# Autodesk Inventor assembly: Clutch Concept
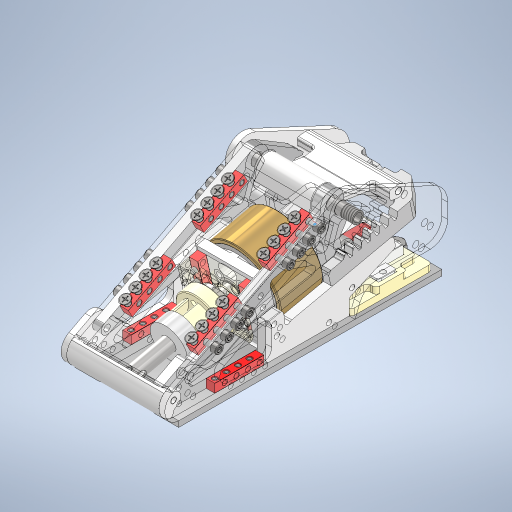
[picture p0: Inventor's stored thumbnail of the model, 512x512]
Saved by Autodesk Inventor 2023.4 (Build 274418000, 418)
## iProperties
Created: 2024-02-03
Part Number: Clutch Concept
Document SubType Name: Assembly
Designer: Nathan Cai
Mass: 541.92 g
Surface Area: 1727.46 cm^2
Volume: 204.134 cm^3
Density: 2.65472 g/cm^3
Author: Nathan Cai
## Documents named in this file (42)
- E:\Documents\Inventor\Bleep V1.2\Clutch Concept.iam
- E:\Documents\Inventor\Bleep V1.2\Flywheel.ipt
- E:\Documents\Inventor\Bleep V1.2\Thrust Bearing.ipt
- E:\Documents\Inventor\Bleep V1.2\BB 13x19x4.ipt
- E:\Documents\Inventor\Bleep V1.2\Cup.ipt
- E:\Documents\Inventor\Bleep V1.2\1561T741_Stacked Wave Disc Spring\1561T741_Stacked Wave Disc Spring.ipt
- E:\Documents\Inventor\Bleep V1.2\AKK RS2205 2300KV\AKK RS2205 2300KV.iam
- E:\Documents\Inventor\Bleep V1.2\Nut Strip 2x1 - 4-40.ipt
- E:\Documents\Inventor\Bleep V1.2\BB 37mm x 30mm x 4mm.ipt
- E:\Documents\Inventor\Bleep V1.2\Motor Plate.ipt
- E:\Documents\Inventor\Bleep V1.2\Uprights.ipt
- E:\Documents\Inventor\Bleep V1.2\Nut Strip 4x4 - 4-40.ipt
- E:\Documents\Inventor\Bleep V1.2\5172T23_Metal Gear - 20 Degree Pressure Angle\5172T23_Metal Gear - 20 Degree Pressure Angle.ipt
- E:\Documents\Inventor\Bleep V1.2\BB .25x.5x.1875 - Flangeless.ipt
- E:\Documents\Inventor\Content Center Files\R2023\en-US\ANSI B18.3(13)\ANSI B18.3 - 4-40 UNC - 0.375(22).ipt
- E:\Documents\Inventor\Bleep V1.2\Lever.ipt
- E:\Documents\Inventor\Bleep V1.2\Servo Support.ipt
- E:\Documents\Inventor\Bleep V1.2\Part1\Part1.ipt
- E:\Documents\Inventor\Bleep V1.2\Cam - Lever.ipt
- E:\Documents\Inventor\Bleep V1.2\Cam - Shell.ipt
- E:\Documents\Inventor\Bleep V1.2\BB 3x7x3.ipt
- E:\Documents\Inventor\Bleep V1.2\Ramp.ipt
- E:\Documents\Inventor\Bleep V1.2\Lever - Copy.ipt
- E:\Documents\Inventor\Bleep V1.2\Brace.ipt
- E:\Documents\Inventor\Bleep V1.2\BB 3x7x3 - Copy.ipt
- E:\Documents\Inventor\Bleep V1.2\Shaft - Arms.ipt
- E:\Documents\Inventor\Bleep V1.2\Shaft - Flywheel C.ipt
- E:\Documents\Inventor\Bleep V1.2\Clutch C.ipt
- E:\Documents\Inventor\Bleep V1.2\Spring Mount.ipt
- E:\Documents\Inventor\Bleep V1.2\Spring Spool.ipt
- E:\Documents\Inventor\Bleep V1.2\Collar.ipt
- E:\Documents\Inventor\Bleep V1.2\Bottom Plate.ipt
- E:\Documents\Inventor\Content Center Files\R2023\en-US\ANSI B18.6.3(12)\ANSI B18.6.3 - 4-40 UNC - 0.375(15_).ipt
- E:\Documents\Inventor\Bleep V1.2\Crown.ipt
- E:\Documents\Inventor\Bleep V1.2\Front Bumper.ipt
- E:\Documents\Inventor\Content Center Files\R2023\en-US\ANSI B18.6.3(12)\ANSI B18.6.3 - 4-40 UNC - 0.3125(15_).ipt
- E:\Documents\Inventor\Content Center Files\R2023\en-US\ANSI B18.6.3(12)\ANSI B18.6.3 - 6-32 UNC - 0.375(15_).ipt
- E:\Documents\Inventor\Content Center Files\R2023\en-US\ANSI B18.2.2(06)\ANSI B18.2.2 - 6 - 32(06).ipt
- E:\Documents\Inventor\Content Center Files\R2023\en-US\ANSI B18.6.3(14)\ANSI B18.6.3 - 6-32 UNC - 0.625(6).ipt
- E:\Documents\Inventor\Bleep V1.2\Rack - Slot.ipt
- E:\Documents\Inventor\Bleep V1.2\Export\STL\Lever Spacer.ipt
- E:\Documents\Inventor\Bleep V1.2\Uprights- Exterior.ipt
## Components (110 placed, 41 different names)
1. Front Bumper:1 — Angle:5
2. Bottom Plate:1 — Mate:347, Flush:153, Mate:402, Mate:403, Mate:404, Mate:405, Mate:406, Mate:407, Mate:408, Mate:409, Mate:410, Mate:411, Mate:412, Mate:413, Mate:414, Mate:415, Mate:416, Mate:417, Mate:418, Mate:420, Mate:422, Mate:424
3. Crown:1 — Mate:386, Mate:387
4. Lever Spacer:1 — Mate:462, Mate:463
5. Uprights- Exterior:1 — Mate:470, Mate:471, Mate:472
6. Uprights- Exterior:2 — Mate:473, Mate:474, Mate:475
7. Flywheel:1 — Mate:37, Flush:102, Mate:104, Mate:105, Mate:275, Mate:309
8. Shaft - Flywheel C:1 — Mate:306, Mate:307, Mate:308, Mate:310, Mate:311, Mate:312, Mate:313, Mate:314, Mate:315, Angle:4, Mate:319, Mate:321, Mate:324
9. Shaft - Arms:1 — Mate:257, Flush:118, Mate:386, Mate:471, Mate:474
10. Clutch C:1 — Mate:308, Angle:4
11. Rack - Slot:1 — Angle:1, Angle:3, Rotation/Translation:1, Mate:315, Mate:313, Mate:314
12. Cup:1 — Mate:26, Mate:27, Angle:1, Tangent:1
13. AKK RS2205 2300KV:1 [sub-assembly] — Mate:37, Flush:102, Mate:426
14. Motor Plate:1 — Mate:106, Mate:107, Mate:128, Mate:129, Mate:131, Mate:132, Mate:134, Mate:136, Flush:106, Mate:144, Mate:145, Mate:146, Mate:147, Mate:148, Mate:149, Mate:150, Mate:151, Mate:152, Mate:153, Mate:154, Mate:155, Mate:156, Mate:157, Mate:158, Mate:159, Flush:149, Mate:426
15. 1561T741_Stacked Wave Disc Spring:1 — Mate:311, Mate:312
16. Spring Mount:1 — Mate:316, Flush:149, Mate:317, Mate:320
17. Thrust Bearing:1 — Mate:319, Mate:320, Mate:322
18. Spring Spool:1 — Mate:321, Mate:322, Mate:325
19. Collar:1 — Mate:324, Mate:325
20. Uprights:1 — Mate:128, Mate:130, Flush:103, Flush:104, Mate:133, Mate:138, Mate:141, Flush:107, Mate:168, Mate:169, Flush:108, Mate:229, Mate:230, Flush:110, Mate:257, Mate:266, Mate:267, Mate:268, Mate:269, Flush:125, Mate:317, Mate:289, Mate:347, Mate:363
21. Uprights:2 — Flush:103, Mate:132, Flush:104, Mate:135, Mate:137, Mate:139, Mate:140, Mate:191, Mate:226, Mate:228, Flush:111, Mate:263, Mate:264, Mate:270, Mate:271, Flush:124, Mate:292, Mate:362, Mate:387, Angle:5
22. Brace:1 — Mate:226, Mate:228, Flush:111, Mate:292, Mate:470
23. Brace:2 — Mate:229, Mate:230, Flush:110, Mate:289, Mate:473
24. Nut Strip 4x4 - 4-40:1 — Mate:129, Mate:130, Mate:131, Mate:133, Mate:316
25. Nut Strip 4x4 - 4-40:2 — Mate:134, Mate:135, Mate:136, Mate:137
26. 5172T23_Metal Gear - 20 Degree Pressure Angle:1 — Mate:138, Mate:141, Flush:105, Angle:3, Mate:198, Mate:199, Mate:200, Mate:201, Mate:202, Mate:203, Mate:204, Rotation/Translation:1, Flush:118, Mate:369, Mate:427, Mate:428, Mate:429, Mate:430, Mate:431, Mate:432, Mate:433, Mate:434, Mate:435, Mate:436, Mate:437, Mate:438, Mate:439, Mate:440, Mate:441, Mate:442
27. 5172T23_Metal Gear - 20 Degree Pressure Angle:2 — Mate:139, Mate:140, Flush:105, Mate:192, Mate:193, Mate:194, Mate:195, Mate:196, Mate:197, Flush:150, Mate:443, Mate:444, Mate:445, Mate:446, Mate:447, Mate:448, Mate:449, Mate:450, Mate:451, Mate:452, Mate:453, Mate:454, Mate:455, Mate:456, Mate:457, Mate:458
28. BB .25x.5x.1875 - Flangeless:1 — Flush:106, Mate:310
29. Lever:1 — Mate:168, Mate:169, Tangent:1, Mate:181, Mate:182, Mate:190, Mate:326, Mate:327
30. Lever - Copy:1
31. Part1:1 — Mate:179, Mate:180, Mate:186, Mate:187, Mate:188
32. Cam - Lever:1 — Mate:177, Mate:178, Mate:327
33. Cam - Shell:1 — Mate:177, Mate:178, Mate:179, Mate:180
34. BB 3x7x3:1 — Mate:181, Mate:182
35. BB 3x7x3:2 — Mate:462, Mate:463
36. BB 3x7x3 - Copy:1 — Mate:190, Mate:326
37. BB 13x19x4:1 — Mate:26, Mate:27
38. BB 37mm x 30mm x 4mm:1 — Mate:104, Mate:105, Mate:106, Mate:107
39. BB .25x.5x.1875 - Flangeless:2 — Mate:275, Mate:306, Mate:307, Mate:309
40. Servo Support:1 — Mate:186, Mate:187, Mate:188, Flush:108, Mate:191, Flush:153, Mate:419, Mate:421, Mate:423, Mate:425
41. Ramp:1 — Mate:204, Flush:150, Mate:369, Mate:370, Mate:371, Mate:372, Mate:373, Mate:374, Mate:375, Mate:376, Mate:377, Mate:378, Mate:379, Mate:380, Mate:381, Mate:382, Mate:383, Mate:384, Mate:385
42. Nut Strip 4x4 - 4-40:3 — Mate:192, Mate:193, Mate:194
43. Nut Strip 4x4 - 4-40:5 — Mate:199, Mate:200, Mate:201
44. Nut Strip 4x4 - 4-40:6 — Mate:198, Mate:202, Mate:203
45. Nut Strip 4x4 - 4-40:7 — Mate:195, Mate:196, Mate:197
46. Nut Strip 4x4 - 4-40:8 — Mate:266, Mate:267, Mate:363, Mate:475
47. Nut Strip 4x4 - 4-40:9 — Mate:263, Mate:264, Mate:362, Mate:472
48. Nut Strip 2x1 - 4-40:3 — Mate:270, Mate:271, Flush:124
49. Nut Strip 2x1 - 4-40:4 — Mate:268, Mate:269, Flush:125
50. Cross Recessed Flat Countersunk Head Machine Screw - Type II - Inch 6-32 x 5/8:1
51. Spline Socket Head Cap Screw - Inch 4-40 UNC - 0.375:9 — Mate:427, Mate:428
52. Spline Socket Head Cap Screw - Inch 4-40 UNC - 0.375:10 — Mate:429, Mate:430
53. Spline Socket Head Cap Screw - Inch 4-40 UNC - 0.375:11 — Mate:431, Mate:432
54. Spline Socket Head Cap Screw - Inch 4-40 UNC - 0.375:12 — Mate:433, Mate:434
55. Spline Socket Head Cap Screw - Inch 4-40 UNC - 0.375:13 — Mate:435, Mate:436
56. Spline Socket Head Cap Screw - Inch 4-40 UNC - 0.375:14 — Mate:437, Mate:438
57. Spline Socket Head Cap Screw - Inch 4-40 UNC - 0.375:15 — Mate:439, Mate:440
58. Spline Socket Head Cap Screw - Inch 4-40 UNC - 0.375:16 — Mate:441, Mate:442
59. Spline Socket Head Cap Screw - Inch 4-40 UNC - 0.375:17 — Mate:443, Mate:444
60. Spline Socket Head Cap Screw - Inch 4-40 UNC - 0.375:18 — Mate:445, Mate:446
61. Spline Socket Head Cap Screw - Inch 4-40 UNC - 0.375:19 — Mate:447, Mate:448
62. Spline Socket Head Cap Screw - Inch 4-40 UNC - 0.375:20 — Mate:449, Mate:450
63. Spline Socket Head Cap Screw - Inch 4-40 UNC - 0.375:21 — Mate:451, Mate:452
64. Spline Socket Head Cap Screw - Inch 4-40 UNC - 0.375:22 — Mate:453, Mate:454
65. Spline Socket Head Cap Screw - Inch 4-40 UNC - 0.375:23 — Mate:455, Mate:456
66. Spline Socket Head Cap Screw - Inch 4-40 UNC - 0.375:24 — Mate:457, Mate:458
67. Cross Recessed Flat Countersunk Head Machine Screw - Type I - Inch 4-40 x 5/16:1 — Mate:402
68. Cross Recessed Flat Countersunk Head Machine Screw - Type I - Inch 4-40 x 5/16:2 — Mate:403
69. Cross Recessed Flat Countersunk Head Machine Screw - Type I - Inch 4-40 x 5/16:3 — Mate:404
70. Cross Recessed Flat Countersunk Head Machine Screw - Type I - Inch 4-40 x 5/16:4 — Mate:405
71. Cross Recessed Flat Countersunk Head Machine Screw - Type I - Inch 4-40 x 5/16:5 — Mate:406
72. Cross Recessed Flat Countersunk Head Machine Screw - Type I - Inch 4-40 x 5/16:6 — Mate:407
73. Cross Recessed Flat Countersunk Head Machine Screw - Type I - Inch 4-40 x 5/16:7 — Mate:408
74. Cross Recessed Flat Countersunk Head Machine Screw - Type I - Inch 4-40 x 5/16:8 — Mate:409
75. Cross Recessed Flat Countersunk Head Machine Screw - Type I - Inch 4-40 x 5/16:9 — Mate:410
76. Cross Recessed Flat Countersunk Head Machine Screw - Type I - Inch 4-40 x 5/16:10 — Mate:411
77. Cross Recessed Flat Countersunk Head Machine Screw - Type I - Inch 4-40 x 5/16:11 — Mate:412
78. Cross Recessed Flat Countersunk Head Machine Screw - Type I - Inch 4-40 x 5/16:12 — Mate:413
79. Cross Recessed Flat Countersunk Head Machine Screw - Type I - Inch 6-32 x 3/8:1 — Mate:414
80. Hex Machine Screw Nut - Inch 6 - 32:1 — Mate:418, Mate:419
81. Cross Recessed Flat Countersunk Head Machine Screw - Type I - Inch 6-32 x 3/8:2 — Mate:415
82. Cross Recessed Flat Countersunk Head Machine Screw - Type I - Inch 6-32 x 3/8:3 — Mate:416
83. Cross Recessed Flat Countersunk Head Machine Screw - Type I - Inch 6-32 x 3/8:4 — Mate:417
84. Hex Machine Screw Nut - Inch 6 - 32:2 — Mate:420, Mate:421
85. Hex Machine Screw Nut - Inch 6 - 32:3 — Mate:422, Mate:423
86. Hex Machine Screw Nut - Inch 6 - 32:4 — Mate:424, Mate:425
87. Cross Recessed Flat Countersunk Head Machine Screw - Type I - Inch 4-40 x 3/8:1 — Mate:370
88. Cross Recessed Flat Countersunk Head Machine Screw - Type I - Inch 4-40 x 3/8:2 — Mate:371
89. Cross Recessed Flat Countersunk Head Machine Screw - Type I - Inch 4-40 x 3/8:3 — Mate:372
90. Cross Recessed Flat Countersunk Head Machine Screw - Type I - Inch 4-40 x 3/8:4 — Mate:373
91. Cross Recessed Flat Countersunk Head Machine Screw - Type I - Inch 4-40 x 3/8:5 — Mate:374
92. Cross Recessed Flat Countersunk Head Machine Screw - Type I - Inch 4-40 x 3/8:6 — Mate:375
93. Cross Recessed Flat Countersunk Head Machine Screw - Type I - Inch 4-40 x 3/8:7 — Mate:376
94. Cross Recessed Flat Countersunk Head Machine Screw - Type I - Inch 4-40 x 3/8:8 — Mate:377
95. Cross Recessed Flat Countersunk Head Machine Screw - Type I - Inch 4-40 x 3/8:9 — Mate:378
96. Cross Recessed Flat Countersunk Head Machine Screw - Type I - Inch 4-40 x 3/8:10 — Mate:379
97. Cross Recessed Flat Countersunk Head Machine Screw - Type I - Inch 4-40 x 3/8:11 — Mate:380
98. Cross Recessed Flat Countersunk Head Machine Screw - Type I - Inch 4-40 x 3/8:12 — Mate:381
99. Cross Recessed Flat Countersunk Head Machine Screw - Type I - Inch 4-40 x 3/8:13 — Mate:382
100. Cross Recessed Flat Countersunk Head Machine Screw - Type I - Inch 4-40 x 3/8:14 — Mate:383
101. Cross Recessed Flat Countersunk Head Machine Screw - Type I - Inch 4-40 x 3/8:15 — Mate:384
102. Cross Recessed Flat Countersunk Head Machine Screw - Type I - Inch 4-40 x 3/8:16 — Mate:385
103. Spline Socket Head Cap Screw - Inch 4-40 UNC - 0.375:1 — Mate:144, Mate:145
104. Spline Socket Head Cap Screw - Inch 4-40 UNC - 0.375:2 — Mate:146, Mate:147
105. Spline Socket Head Cap Screw - Inch 4-40 UNC - 0.375:3 — Mate:148, Mate:149
106. Spline Socket Head Cap Screw - Inch 4-40 UNC - 0.375:4 — Mate:150, Mate:151
107. Spline Socket Head Cap Screw - Inch 4-40 UNC - 0.375:5 — Mate:152, Mate:153
108. Spline Socket Head Cap Screw - Inch 4-40 UNC - 0.375:6 — Mate:154, Mate:155
109. Spline Socket Head Cap Screw - Inch 4-40 UNC - 0.375:7 — Mate:156, Mate:157
110. Spline Socket Head Cap Screw - Inch 4-40 UNC - 0.375:8 — Mate:158, Mate:159
## Relationships (214: Mate 193, Flush 15, Angle 4, Tangent 1, RelateRotateTranslate 1)
- [Mate]: Clutch C:1 ↔ BB 13x19x4:1
- [Mate]: Clutch C:1 ↔ BB 13x19x4:1
- Mate:26: Cup:1 ↔ BB 13x19x4:1
- Mate:27: Cup:1 ↔ BB 13x19x4:1
- Mate:37: Flywheel:1 ↔ AKK RS2205 2300KV:1
- Angle:1 (0 deg): Rack - Slot:1 ↔ Cup:1
- Flush:102: Flywheel:1 ↔ AKK RS2205 2300KV:1
- Mate:104: Flywheel:1 ↔ BB 37mm x 30mm x 4mm:1
- Mate:105: Flywheel:1 ↔ BB 37mm x 30mm x 4mm:1
- Mate:106: Motor Plate:1 ↔ BB 37mm x 30mm x 4mm:1
- Mate:107: Motor Plate:1 ↔ BB 37mm x 30mm x 4mm:1
- Mate:128: Motor Plate:1 ↔ Uprights:1
- Mate:129: Motor Plate:1 ↔ Nut Strip 4x4 - 4-40:1
- Mate:130: Uprights:1 ↔ Nut Strip 4x4 - 4-40:1
- Mate:131: Motor Plate:1 ↔ Nut Strip 4x4 - 4-40:1
- Flush:103: Uprights:1 ↔ Uprights:2
- Mate:132: Motor Plate:1 ↔ Uprights:2
- Flush:104: Uprights:1 ↔ Uprights:2
- Mate:133: Uprights:1 ↔ Nut Strip 4x4 - 4-40:1
- Mate:134: Motor Plate:1 ↔ Nut Strip 4x4 - 4-40:2
- Mate:135: Uprights:2 ↔ Nut Strip 4x4 - 4-40:2
- Mate:136: Motor Plate:1 ↔ Nut Strip 4x4 - 4-40:2
- Mate:137: Uprights:2 ↔ Nut Strip 4x4 - 4-40:2
- Mate:138: Uprights:1 ↔ 5172T23_Metal Gear - 20 Degree Pressure Angle:1
- Mate:139: Uprights:2 ↔ 5172T23_Metal Gear - 20 Degree Pressure Angle:2
- Mate:140: Uprights:2 ↔ 5172T23_Metal Gear - 20 Degree Pressure Angle:2
- Mate:141: Uprights:1 ↔ 5172T23_Metal Gear - 20 Degree Pressure Angle:1
- Flush:105: 5172T23_Metal Gear - 20 Degree Pressure Angle:1 ↔ 5172T23_Metal Gear - 20 Degree Pressure Angle:2
- Flush:106: Motor Plate:1 ↔ BB .25x.5x.1875 - Flangeless:1
- Mate:144: Motor Plate:1 ↔ Spline Socket Head Cap Screw - Inch 4-40 UNC - 0.375:1
- Mate:145: Motor Plate:1 ↔ Spline Socket Head Cap Screw - Inch 4-40 UNC - 0.375:1
- Mate:146: Motor Plate:1 ↔ Spline Socket Head Cap Screw - Inch 4-40 UNC - 0.375:2
- Mate:147: Motor Plate:1 ↔ Spline Socket Head Cap Screw - Inch 4-40 UNC - 0.375:2
- Mate:148: Motor Plate:1 ↔ Spline Socket Head Cap Screw - Inch 4-40 UNC - 0.375:3
- Mate:149: Motor Plate:1 ↔ Spline Socket Head Cap Screw - Inch 4-40 UNC - 0.375:3
- Mate:150: Motor Plate:1 ↔ Spline Socket Head Cap Screw - Inch 4-40 UNC - 0.375:4
- Mate:151: Motor Plate:1 ↔ Spline Socket Head Cap Screw - Inch 4-40 UNC - 0.375:4
- Mate:152: Motor Plate:1 ↔ Spline Socket Head Cap Screw - Inch 4-40 UNC - 0.375:5
- Mate:153: Motor Plate:1 ↔ Spline Socket Head Cap Screw - Inch 4-40 UNC - 0.375:5
- Mate:154: Motor Plate:1 ↔ Spline Socket Head Cap Screw - Inch 4-40 UNC - 0.375:6
- Mate:155: Motor Plate:1 ↔ Spline Socket Head Cap Screw - Inch 4-40 UNC - 0.375:6
- Mate:156: Motor Plate:1 ↔ Spline Socket Head Cap Screw - Inch 4-40 UNC - 0.375:7
- Mate:157: Motor Plate:1 ↔ Spline Socket Head Cap Screw - Inch 4-40 UNC - 0.375:7
- Mate:158: Motor Plate:1 ↔ Spline Socket Head Cap Screw - Inch 4-40 UNC - 0.375:8
- Mate:159: Motor Plate:1 ↔ Spline Socket Head Cap Screw - Inch 4-40 UNC - 0.375:8
- Flush:107: Uprights:1
- Mate:168: Uprights:1 ↔ Lever:1
- Mate:169: Uprights:1 ↔ Lever:1
- Tangent:1: Cup:1 ↔ Lever:1
- Angle:3 (0 deg): Rack - Slot:1 ↔ 5172T23_Metal Gear - 20 Degree Pressure Angle:1
- [Mate]: Uprights:2 ↔ Lever - Copy:1
- [Mate]: Uprights:2 ↔ Lever - Copy:1
- [Mate]: Lever:1 ↔ Lever - Copy:1
- Mate:177: Cam - Lever:1 ↔ Cam - Shell:1
- Mate:178: Cam - Lever:1 ↔ Cam - Shell:1
- Mate:179: Part1:1 ↔ Cam - Shell:1
- Mate:180: Part1:1 ↔ Cam - Shell:1
- Mate:181: Lever:1 ↔ BB 3x7x3:1
- Mate:182: Lever:1 ↔ BB 3x7x3:1
- [Mate]: Lever - Copy:1 ↔ BB 3x7x3:2
- [Mate]: Lever - Copy:1 ↔ BB 3x7x3:2
- Mate:186: Part1:1 ↔ Servo Support:1
- Mate:187: Part1:1 ↔ Servo Support:1
- Mate:188: Part1:1 ↔ Servo Support:1
- Flush:108: Uprights:1 ↔ Servo Support:1
- Mate:190: Lever:1 ↔ BB 3x7x3 - Copy:1
- Mate:191: Uprights:2 ↔ Servo Support:1
- Mate:192: 5172T23_Metal Gear - 20 Degree Pressure Angle:2 ↔ Nut Strip 4x4 - 4-40:3
- Mate:193: 5172T23_Metal Gear - 20 Degree Pressure Angle:2 ↔ Nut Strip 4x4 - 4-40:3
- Mate:194: 5172T23_Metal Gear - 20 Degree Pressure Angle:2 ↔ Nut Strip 4x4 - 4-40:3
- Mate:195: 5172T23_Metal Gear - 20 Degree Pressure Angle:2 ↔ Nut Strip 4x4 - 4-40:7
- Mate:196: 5172T23_Metal Gear - 20 Degree Pressure Angle:2 ↔ Nut Strip 4x4 - 4-40:7
- Mate:197: 5172T23_Metal Gear - 20 Degree Pressure Angle:2 ↔ Nut Strip 4x4 - 4-40:7
- Mate:198: 5172T23_Metal Gear - 20 Degree Pressure Angle:1 ↔ Nut Strip 4x4 - 4-40:6
- Mate:199: 5172T23_Metal Gear - 20 Degree Pressure Angle:1 ↔ Nut Strip 4x4 - 4-40:5
- Mate:200: 5172T23_Metal Gear - 20 Degree Pressure Angle:1 ↔ Nut Strip 4x4 - 4-40:5
- Mate:201: 5172T23_Metal Gear - 20 Degree Pressure Angle:1 ↔ Nut Strip 4x4 - 4-40:5
- Mate:202: 5172T23_Metal Gear - 20 Degree Pressure Angle:1 ↔ Nut Strip 4x4 - 4-40:6
- Mate:203: 5172T23_Metal Gear - 20 Degree Pressure Angle:1 ↔ Nut Strip 4x4 - 4-40:6
- Mate:204: 5172T23_Metal Gear - 20 Degree Pressure Angle:1 ↔ Ramp:1
- Flush:150: 5172T23_Metal Gear - 20 Degree Pressure Angle:2 ↔ Ramp:1
- Mate:226: Uprights:2 ↔ Brace:1
- Mate:228: Uprights:2 ↔ Brace:1
- Mate:229: Uprights:1 ↔ Brace:2
- Mate:230: Uprights:1 ↔ Brace:2
- Rotation/Translation:1 [RelateRotateTranslate] (159.5929 mm): Rack - Slot:1 ↔ 5172T23_Metal Gear - 20 Degree Pressure Angle:1
- Flush:110: Uprights:1 ↔ Brace:2
- Flush:111: Uprights:2 ↔ Brace:1
- Mate:257: Shaft - Arms:1 ↔ Uprights:1
- Flush:118 (-6.35 mm): Shaft - Arms:1 ↔ 5172T23_Metal Gear - 20 Degree Pressure Angle:1
- Mate:315 (31.75 mm): Shaft - Flywheel C:1 ↔ Rack - Slot:1
- Mate:263: Uprights:2 ↔ Nut Strip 4x4 - 4-40:9
- Mate:264: Uprights:2 ↔ Nut Strip 4x4 - 4-40:9
- Mate:266: Uprights:1 ↔ Nut Strip 4x4 - 4-40:8
- Mate:267: Uprights:1 ↔ Nut Strip 4x4 - 4-40:8
- Mate:268: Uprights:1 ↔ Nut Strip 2x1 - 4-40:4
- Mate:269: Uprights:1 ↔ Nut Strip 2x1 - 4-40:4
- Mate:270: Uprights:2 ↔ Nut Strip 2x1 - 4-40:3
- Mate:271: Uprights:2 ↔ Nut Strip 2x1 - 4-40:3
- Flush:124: Uprights:2 ↔ Nut Strip 2x1 - 4-40:3
- Flush:125: Uprights:1 ↔ Nut Strip 2x1 - 4-40:4
- Mate:275: Flywheel:1 ↔ BB .25x.5x.1875 - Flangeless:2
- Mate:289: Uprights:1 ↔ Brace:2
- Mate:292: Uprights:2 ↔ Brace:1
- Mate:306: Shaft - Flywheel C:1 ↔ BB .25x.5x.1875 - Flangeless:2
- Mate:307: Shaft - Flywheel C:1 ↔ BB .25x.5x.1875 - Flangeless:2
- Mate:308: Shaft - Flywheel C:1 ↔ Clutch C:1
- Mate:309: Flywheel:1 ↔ BB .25x.5x.1875 - Flangeless:2
- Mate:310: Shaft - Flywheel C:1 ↔ BB .25x.5x.1875 - Flangeless:1
- Mate:311: Shaft - Flywheel C:1 ↔ 1561T741_Stacked Wave Disc Spring:1
- Mate:312: Shaft - Flywheel C:1 ↔ 1561T741_Stacked Wave Disc Spring:1
- Mate:313: Shaft - Flywheel C:1 ↔ Rack - Slot:1
- Mate:314: Shaft - Flywheel C:1 ↔ Rack - Slot:1
- Angle:4 (0 deg): Shaft - Flywheel C:1 ↔ Clutch C:1
- Mate:316: Spring Mount:1 ↔ Nut Strip 4x4 - 4-40:1
- Flush:149 (2.3813 mm): Motor Plate:1 ↔ Spring Mount:1
- Mate:317: Spring Mount:1 ↔ Uprights:1
- Mate:319: Shaft - Flywheel C:1 ↔ Thrust Bearing:1
- Mate:320: Spring Mount:1 ↔ Thrust Bearing:1
- Mate:321: Shaft - Flywheel C:1 ↔ Spring Spool:1
- Mate:322: Thrust Bearing:1 ↔ Spring Spool:1
- Mate:324: Shaft - Flywheel C:1 ↔ Collar:1
- Mate:325: Spring Spool:1 ↔ Collar:1
- Mate:326: Lever:1 ↔ BB 3x7x3 - Copy:1
- Mate:327: Lever:1 ↔ Cam - Lever:1
- Mate:347: Bottom Plate:1 ↔ Uprights:1
- Flush:153 (-3.175 mm): Bottom Plate:1 ↔ Servo Support:1
- Mate:362: Uprights:2 ↔ Nut Strip 4x4 - 4-40:9
- Mate:363: Uprights:1 ↔ Nut Strip 4x4 - 4-40:8
- Mate:369: 5172T23_Metal Gear - 20 Degree Pressure Angle:1 ↔ Ramp:1
- Mate:370: Ramp:1 ↔ Cross Recessed Flat Countersunk Head Machine Screw - Type I - Inch 4-40 x 3/8:1
- Mate:371: Ramp:1 ↔ Cross Recessed Flat Countersunk Head Machine Screw - Type I - Inch 4-40 x 3/8:2
- Mate:372: Ramp:1 ↔ Cross Recessed Flat Countersunk Head Machine Screw - Type I - Inch 4-40 x 3/8:3
- Mate:373: Ramp:1 ↔ Cross Recessed Flat Countersunk Head Machine Screw - Type I - Inch 4-40 x 3/8:4
- Mate:374: Ramp:1 ↔ Cross Recessed Flat Countersunk Head Machine Screw - Type I - Inch 4-40 x 3/8:5
- Mate:375: Ramp:1 ↔ Cross Recessed Flat Countersunk Head Machine Screw - Type I - Inch 4-40 x 3/8:6
- Mate:376: Ramp:1 ↔ Cross Recessed Flat Countersunk Head Machine Screw - Type I - Inch 4-40 x 3/8:7
- Mate:377: Ramp:1 ↔ Cross Recessed Flat Countersunk Head Machine Screw - Type I - Inch 4-40 x 3/8:8
- Mate:378: Ramp:1 ↔ Cross Recessed Flat Countersunk Head Machine Screw - Type I - Inch 4-40 x 3/8:9
- Mate:379: Ramp:1 ↔ Cross Recessed Flat Countersunk Head Machine Screw - Type I - Inch 4-40 x 3/8:10
- Mate:380: Ramp:1 ↔ Cross Recessed Flat Countersunk Head Machine Screw - Type I - Inch 4-40 x 3/8:11
- Mate:381: Ramp:1 ↔ Cross Recessed Flat Countersunk Head Machine Screw - Type I - Inch 4-40 x 3/8:12
- Mate:382: Ramp:1 ↔ Cross Recessed Flat Countersunk Head Machine Screw - Type I - Inch 4-40 x 3/8:13
- Mate:383: Ramp:1 ↔ Cross Recessed Flat Countersunk Head Machine Screw - Type I - Inch 4-40 x 3/8:14
- Mate:384: Ramp:1 ↔ Cross Recessed Flat Countersunk Head Machine Screw - Type I - Inch 4-40 x 3/8:15
- Mate:385: Ramp:1 ↔ Cross Recessed Flat Countersunk Head Machine Screw - Type I - Inch 4-40 x 3/8:16
- Mate:386: Crown:1 ↔ Shaft - Arms:1
- Mate:387: Crown:1 ↔ Uprights:2
- Angle:5 (180 deg): Front Bumper:1 ↔ Uprights:2
- Mate:402: Bottom Plate:1 ↔ Cross Recessed Flat Countersunk Head Machine Screw - Type I - Inch 4-40 x 5/16:1
- Mate:403: Bottom Plate:1 ↔ Cross Recessed Flat Countersunk Head Machine Screw - Type I - Inch 4-40 x 5/16:2
- Mate:404: Bottom Plate:1 ↔ Cross Recessed Flat Countersunk Head Machine Screw - Type I - Inch 4-40 x 5/16:3
- Mate:405: Bottom Plate:1 ↔ Cross Recessed Flat Countersunk Head Machine Screw - Type I - Inch 4-40 x 5/16:4
- Mate:406: Bottom Plate:1 ↔ Cross Recessed Flat Countersunk Head Machine Screw - Type I - Inch 4-40 x 5/16:5
- Mate:407: Bottom Plate:1 ↔ Cross Recessed Flat Countersunk Head Machine Screw - Type I - Inch 4-40 x 5/16:6
- Mate:408: Bottom Plate:1 ↔ Cross Recessed Flat Countersunk Head Machine Screw - Type I - Inch 4-40 x 5/16:7
- Mate:409: Bottom Plate:1 ↔ Cross Recessed Flat Countersunk Head Machine Screw - Type I - Inch 4-40 x 5/16:8
- Mate:410: Bottom Plate:1 ↔ Cross Recessed Flat Countersunk Head Machine Screw - Type I - Inch 4-40 x 5/16:9
- Mate:411: Bottom Plate:1 ↔ Cross Recessed Flat Countersunk Head Machine Screw - Type I - Inch 4-40 x 5/16:10
- Mate:412: Bottom Plate:1 ↔ Cross Recessed Flat Countersunk Head Machine Screw - Type I - Inch 4-40 x 5/16:11
- Mate:413: Bottom Plate:1 ↔ Cross Recessed Flat Countersunk Head Machine Screw - Type I - Inch 4-40 x 5/16:12
- Mate:414: Bottom Plate:1 ↔ Cross Recessed Flat Countersunk Head Machine Screw - Type I - Inch 6-32 x 3/8:1
- Mate:415: Bottom Plate:1 ↔ Cross Recessed Flat Countersunk Head Machine Screw - Type I - Inch 6-32 x 3/8:2
- Mate:416: Bottom Plate:1 ↔ Cross Recessed Flat Countersunk Head Machine Screw - Type I - Inch 6-32 x 3/8:3
- Mate:417: Bottom Plate:1 ↔ Cross Recessed Flat Countersunk Head Machine Screw - Type I - Inch 6-32 x 3/8:4
- Mate:418: Bottom Plate:1 ↔ Hex Machine Screw Nut - Inch 6 - 32:1
- Mate:419: Servo Support:1 ↔ Hex Machine Screw Nut - Inch 6 - 32:1
- Mate:420: Bottom Plate:1 ↔ Hex Machine Screw Nut - Inch 6 - 32:2
- Mate:421: Servo Support:1 ↔ Hex Machine Screw Nut - Inch 6 - 32:2
- Mate:422: Bottom Plate:1 ↔ Hex Machine Screw Nut - Inch 6 - 32:3
- Mate:423: Servo Support:1 ↔ Hex Machine Screw Nut - Inch 6 - 32:3
- Mate:424: Bottom Plate:1 ↔ Hex Machine Screw Nut - Inch 6 - 32:4
- Mate:425: Servo Support:1 ↔ Hex Machine Screw Nut - Inch 6 - 32:4
- Mate:426: AKK RS2205 2300KV:1 ↔ Motor Plate:1
- Mate:427: 5172T23_Metal Gear - 20 Degree Pressure Angle:1 ↔ Spline Socket Head Cap Screw - Inch 4-40 UNC - 0.375:9
- Mate:428: 5172T23_Metal Gear - 20 Degree Pressure Angle:1 ↔ Spline Socket Head Cap Screw - Inch 4-40 UNC - 0.375:9
- Mate:429: 5172T23_Metal Gear - 20 Degree Pressure Angle:1 ↔ Spline Socket Head Cap Screw - Inch 4-40 UNC - 0.375:10
- Mate:430: 5172T23_Metal Gear - 20 Degree Pressure Angle:1 ↔ Spline Socket Head Cap Screw - Inch 4-40 UNC - 0.375:10
- Mate:431: 5172T23_Metal Gear - 20 Degree Pressure Angle:1 ↔ Spline Socket Head Cap Screw - Inch 4-40 UNC - 0.375:11
- Mate:432: 5172T23_Metal Gear - 20 Degree Pressure Angle:1 ↔ Spline Socket Head Cap Screw - Inch 4-40 UNC - 0.375:11
- Mate:433: 5172T23_Metal Gear - 20 Degree Pressure Angle:1 ↔ Spline Socket Head Cap Screw - Inch 4-40 UNC - 0.375:12
- Mate:434: 5172T23_Metal Gear - 20 Degree Pressure Angle:1 ↔ Spline Socket Head Cap Screw - Inch 4-40 UNC - 0.375:12
- Mate:435: 5172T23_Metal Gear - 20 Degree Pressure Angle:1 ↔ Spline Socket Head Cap Screw - Inch 4-40 UNC - 0.375:13
- Mate:436: 5172T23_Metal Gear - 20 Degree Pressure Angle:1 ↔ Spline Socket Head Cap Screw - Inch 4-40 UNC - 0.375:13
- Mate:437: 5172T23_Metal Gear - 20 Degree Pressure Angle:1 ↔ Spline Socket Head Cap Screw - Inch 4-40 UNC - 0.375:14
- Mate:438: 5172T23_Metal Gear - 20 Degree Pressure Angle:1 ↔ Spline Socket Head Cap Screw - Inch 4-40 UNC - 0.375:14
- Mate:439: 5172T23_Metal Gear - 20 Degree Pressure Angle:1 ↔ Spline Socket Head Cap Screw - Inch 4-40 UNC - 0.375:15
- Mate:440: 5172T23_Metal Gear - 20 Degree Pressure Angle:1 ↔ Spline Socket Head Cap Screw - Inch 4-40 UNC - 0.375:15
- Mate:441: 5172T23_Metal Gear - 20 Degree Pressure Angle:1 ↔ Spline Socket Head Cap Screw - Inch 4-40 UNC - 0.375:16
- Mate:442: 5172T23_Metal Gear - 20 Degree Pressure Angle:1 ↔ Spline Socket Head Cap Screw - Inch 4-40 UNC - 0.375:16
- Mate:443: 5172T23_Metal Gear - 20 Degree Pressure Angle:2 ↔ Spline Socket Head Cap Screw - Inch 4-40 UNC - 0.375:17
- Mate:444: 5172T23_Metal Gear - 20 Degree Pressure Angle:2 ↔ Spline Socket Head Cap Screw - Inch 4-40 UNC - 0.375:17
- Mate:445: 5172T23_Metal Gear - 20 Degree Pressure Angle:2 ↔ Spline Socket Head Cap Screw - Inch 4-40 UNC - 0.375:18
- Mate:446: 5172T23_Metal Gear - 20 Degree Pressure Angle:2 ↔ Spline Socket Head Cap Screw - Inch 4-40 UNC - 0.375:18
- Mate:447: 5172T23_Metal Gear - 20 Degree Pressure Angle:2 ↔ Spline Socket Head Cap Screw - Inch 4-40 UNC - 0.375:19
- Mate:448: 5172T23_Metal Gear - 20 Degree Pressure Angle:2 ↔ Spline Socket Head Cap Screw - Inch 4-40 UNC - 0.375:19
- Mate:449: 5172T23_Metal Gear - 20 Degree Pressure Angle:2 ↔ Spline Socket Head Cap Screw - Inch 4-40 UNC - 0.375:20
- Mate:450: 5172T23_Metal Gear - 20 Degree Pressure Angle:2 ↔ Spline Socket Head Cap Screw - Inch 4-40 UNC - 0.375:20
- Mate:451: 5172T23_Metal Gear - 20 Degree Pressure Angle:2 ↔ Spline Socket Head Cap Screw - Inch 4-40 UNC - 0.375:21
- Mate:452: 5172T23_Metal Gear - 20 Degree Pressure Angle:2 ↔ Spline Socket Head Cap Screw - Inch 4-40 UNC - 0.375:21
- Mate:453: 5172T23_Metal Gear - 20 Degree Pressure Angle:2 ↔ Spline Socket Head Cap Screw - Inch 4-40 UNC - 0.375:22
- Mate:454: 5172T23_Metal Gear - 20 Degree Pressure Angle:2 ↔ Spline Socket Head Cap Screw - Inch 4-40 UNC - 0.375:22
- Mate:455: 5172T23_Metal Gear - 20 Degree Pressure Angle:2 ↔ Spline Socket Head Cap Screw - Inch 4-40 UNC - 0.375:23
- Mate:456: 5172T23_Metal Gear - 20 Degree Pressure Angle:2 ↔ Spline Socket Head Cap Screw - Inch 4-40 UNC - 0.375:23
- Mate:457: 5172T23_Metal Gear - 20 Degree Pressure Angle:2 ↔ Spline Socket Head Cap Screw - Inch 4-40 UNC - 0.375:24
- Mate:458: 5172T23_Metal Gear - 20 Degree Pressure Angle:2 ↔ Spline Socket Head Cap Screw - Inch 4-40 UNC - 0.375:24
- Mate:462: Lever Spacer:1 ↔ BB 3x7x3:2
- Mate:463: Lever Spacer:1 ↔ BB 3x7x3:2
- Mate:470: Uprights- Exterior:1 ↔ Brace:1
- Mate:471: Uprights- Exterior:1 ↔ Shaft - Arms:1
- Mate:472: Uprights- Exterior:1 ↔ Nut Strip 4x4 - 4-40:9
- Mate:473: Uprights- Exterior:2 ↔ Brace:2
- Mate:474: Uprights- Exterior:2 ↔ Shaft - Arms:1
- Mate:475: Uprights- Exterior:2 ↔ Nut Strip 4x4 - 4-40:8
